# Autodesk Inventor assembly: 5WheelAssy
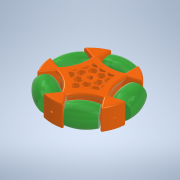
[picture p0: Inventor's stored thumbnail of the model, 180x180]
Saved by Autodesk Inventor 2021 (Build 250183000, 183)
## iProperties
Created: 2023-10-07
Part Number: 5WheelAssy
Document SubType Name: Assembly
Designer: Trey Vokoun
Author: Trey Vokoun
## Documents named in this file (3)
- C:\Users\Trey Vokoun\Documents\Inventor\Doomba\DoombaMk1\OmniWheels\5WheelAssy.iam
- C:\Users\Trey Vokoun\Documents\Inventor\Doomba\DoombaMk1\OmniWheels\5Wheel.ipt
- C:\Users\Trey Vokoun\Documents\Inventor\Doomba\DoombaMk1\OmniWheels\5wheelroller.ipt
## Components (6 placed, 2 different names)
1. 5Wheel:1 — Mate:1, Mate:2, Mate:3, Mate:4, Mate:5, Mate:6, Mate:7, Mate:8, Mate:9, Mate:10
2. 5wheelroller:1 — Mate:1, Mate:6
3. 5wheelroller:2 — Mate:3, Mate:8
4. 5wheelroller:3 — Mate:2, Mate:7
5. 5wheelroller:4 — Mate:4, Mate:9
6. 5wheelroller:5 — Mate:5, Mate:10
## Relationships (10: Mate 10)
- Mate:1: 5Wheel:1 ↔ 5wheelroller:1
- Mate:2: 5Wheel:1 ↔ 5wheelroller:3
- Mate:3: 5Wheel:1 ↔ 5wheelroller:2
- Mate:4: 5Wheel:1 ↔ 5wheelroller:4
- Mate:5: 5Wheel:1 ↔ 5wheelroller:5
- Mate:6: 5Wheel:1 ↔ 5wheelroller:1
- Mate:7: 5Wheel:1 ↔ 5wheelroller:3
- Mate:8: 5Wheel:1 ↔ 5wheelroller:2
- Mate:9: 5Wheel:1 ↔ 5wheelroller:4
- Mate:10: 5Wheel:1 ↔ 5wheelroller:5
